# Autodesk Inventor assembly: 3A.04.01.JS.54mm root_CPY
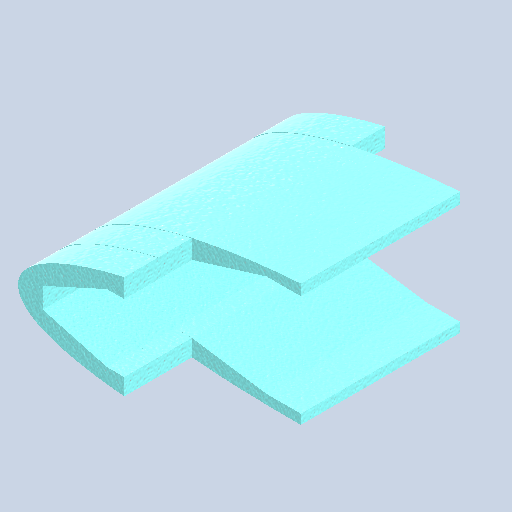
[picture p0: Inventor's stored thumbnail of the model, 512x512]
Saved by Autodesk Inventor 2025.1 (Build 291241000, 241)
## iProperties
Created: 2025-01-14
Part Number: 3A.04.01.JS.54mm root_CPY
Document SubType Name: Assembly
Designer: johan
Author: johan
## Documents named in this file (3)
- C:\Users\johan\OneDrive - University of Bristol\CAD docs\2) Wing\3) Leading edge\assemblies\3A.04.01.JS.54mm root_CPY.iam
- C:\Users\johan\OneDrive - University of Bristol\CAD docs\2) Wing\3) Leading edge\parts\3P.04.01.JS. leading edge 54mm_CPY.ipt
- C:\Users\johan\OneDrive - University of Bristol\CAD docs\2) Wing\3) Leading edge\parts\3P.04.JS.2414 rib leading edge v2_CPY.ipt
## Components (4 placed, 2 different names)
1. 3P.04.01.JS. leading edge 54mm_CPY:1 — Rigid:2, Rigid:1
2. 3P.04.JS.2414 rib leading edge v2_CPY:1 — Rigid:2
3. 3P.04.JS.2414 rib leading edge v2_CPY:2 — Rigid:1, Rigid:3
4. 3P.04.JS.2414 rib leading edge v2_CPY:3 — Rigid:3
## Relationships (3: WeldJoint 3)
- Rigid:2 [WeldJoint]: 3P.04.01.JS. leading edge 54mm_CPY:1 ↔ 3P.04.JS.2414 rib leading edge v2_CPY:1
- Rigid:1 [WeldJoint]: 3P.04.01.JS. leading edge 54mm_CPY:1 ↔ 3P.04.JS.2414 rib leading edge v2_CPY:2
- Rigid:3 [WeldJoint]: 3P.04.JS.2414 rib leading edge v2_CPY:2 ↔ 3P.04.JS.2414 rib leading edge v2_CPY:3
